# Autodesk Inventor assembly: Main_Solar_Structure
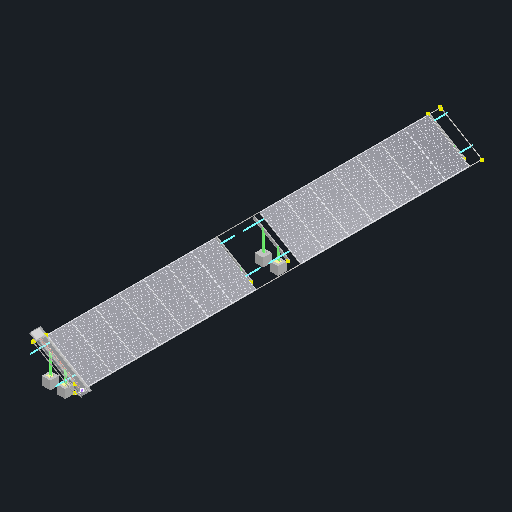
[picture p0: Inventor's stored thumbnail of the model, 512x512]
Saved by Autodesk Inventor 2025.3 (Build 293356030, 356C)
## iProperties
Created: 2019-12-15
Part Number: Main_Solar_Structure
Document SubType Name: Assembly
Designer: Rubens
Sending System: SolidWorks 2021
Last Author: Mohsen
Last Saved: 2022-08-25
Author: Rubens
## Documents named in this file (18)
- C:\Users\Rubens\Downloads\Estrutura Placa - REV00\Solar Mounting Structure\Main_Solar_Structure\Main_Solar_Structure\Estrutura Principal.iam
- C:\Users\Rubens\Downloads\Estrutura Placa - REV00\Solar Mounting Structure\Main_Solar_Structure\Main_Solar_Structure\Small_Column.ipt
- C:\Users\Rubens\Downloads\Estrutura Placa - REV00\Solar Mounting Structure\Main_Solar_Structure\Main_Solar_Structure\Large_Column.ipt
- C:\Users\Rubens\Downloads\Estrutura Placa - REV00\Solar Mounting Structure\Main_Solar_Structure\Main_Solar_Structure\Bottom_Beam.ipt
- C:\Users\Rubens\Downloads\Estrutura Placa - REV00\Solar Mounting Structure\Main_Solar_Structure\Main_Solar_Structure\Top_Beam.iam
- C:\Users\Rubens\Downloads\Estrutura Placa - REV00\Solar Mounting Structure\Main_Solar_Structure\Main_Solar_Structure\Base_Plate.ipt
- C:\Users\Rubens\Downloads\Estrutura Placa - REV00\Solar Mounting Structure\Main_Solar_Structure\Main_Solar_Structure\Base_Support.ipt
- C:\Users\Rubens\Downloads\Estrutura Placa - REV00\Solar Mounting Structure\Main_Solar_Structure\Main_Solar_Structure\Beam_Support.ipt
- C:\Users\Rubens\Downloads\Estrutura Placa - REV00\Solar Mounting Structure\Main_Solar_Structure\Main_Solar_Structure\M10_Screw&Nut.iam
- C:\Users\Rubens\Downloads\Estrutura Placa - REV00\Solar Mounting Structure\Main_Solar_Structure\Main_Solar_Structure\Beam_Connector_Assembly.iam
- C:\Users\Rubens\Downloads\Estrutura Placa - REV00\Solar Mounting Structure\Main_Solar_Structure\Main_Solar_Structure\Base.ipt
- C:\Users\Rubens\Downloads\Estrutura Placa - REV00\Solar Mounting Structure\Main_Solar_Structure\Main_Solar_Structure\ISO - 4034 - M16 - S_.ipt
- C:\Users\Rubens\Downloads\Limpador\MontagemREV0.iam
- C:\Users\Rubens\Downloads\Estrutura Placa - REV00\Solar Mounting Structure\Main_Solar_Structure\Main_Solar_Structure\SolarPV.ipt
- C:\Users\Rubens\Downloads\Estrutura Placa - REV00\Solar Mounting Structure\Main_Solar_Structure\Main_Solar_Structure\Perfil tubo - 30x30x3.ipt
- C:\Users\Rubens\Downloads\Estrutura Placa - REV00\Solar Mounting Structure\Main_Solar_Structure\Main_Solar_Structure\tubo 30 x 30 x 3  - 500.ipt
- C:\Users\Rubens\Downloads\Estrutura Placa - REV00\Solar Mounting Structure\Main_Solar_Structure\Main_Solar_Structure\Limitador.ipt
- C:\Users\Rubens\Downloads\Estrutura Placa - REV00\Solar Mounting Structure\Main_Solar_Structure\Main_Solar_Structure\ISO 12633-2 - 30x30x3 - 2070.ipt
## Components (175 placed, 17 different names)
1. Small_Column:2
2. Base_Plate:2 — Coincidente:15, Coincidente:16, Coincidente:17
3. Base_Plate:4
4. Base_Plate:6
5. Base_Support:3
6. Base_Support:7
7. Base_Support:8
8. Base_Support:9
9. Base_Support:13
10. Base_Support:14
11. Base_Support:15
12. Base_Support:19
13. Base_Support:20
14. Beam_Support:3 — Coincidente:32, Coincidente:33
15. Beam_Support:4 — Coincidente:34, Coincidente:35
16. Beam_Support:5
17. Beam_Support:6
18. Beam_Support:9
19. M10_Screw&Nut:2 [sub-assembly]
20. M10_Screw&Nut:7 [sub-assembly]
21. M10_Screw&Nut:8 [sub-assembly]
22. M10_Screw&Nut:9 [sub-assembly]
23. M10_Screw&Nut:10 [sub-assembly]
24. M10_Screw&Nut:11 [sub-assembly]
25. M10_Screw&Nut:12 [sub-assembly]
26. M10_Screw&Nut:17 [sub-assembly]
27. M10_Screw&Nut:18 [sub-assembly]
28. M10_Screw&Nut:19 [sub-assembly]
29. M10_Screw&Nut:20 [sub-assembly]
30. M10_Screw&Nut:25 [sub-assembly]
31. M10_Screw&Nut:26 [sub-assembly]
32. M10_Screw&Nut:27 [sub-assembly]
33. M10_Screw&Nut:28 [sub-assembly]
34. M10_Screw&Nut:33 [sub-assembly]
35. M10_Screw&Nut:59 [sub-assembly] — Coincidente:63
36. M10_Screw&Nut:60 [sub-assembly]
37. M10_Screw&Nut:61 [sub-assembly]
38. M10_Screw&Nut:62 [sub-assembly]
39. M10_Screw&Nut:63 [sub-assembly]
40. M10_Screw&Nut:64 [sub-assembly]
41. M10_Screw&Nut:65 [sub-assembly]
42. M10_Screw&Nut:66 [sub-assembly]
43. M10_Screw&Nut:67 [sub-assembly]
44. M10_Screw&Nut:68 [sub-assembly]
45. M10_Screw&Nut:69 [sub-assembly]
46. M10_Screw&Nut:71 [sub-assembly] — Coincidente:60
47. M10_Screw&Nut:72 [sub-assembly] — Coincidente:61
48. M10_Screw&Nut:73 [sub-assembly]
49. M10_Screw&Nut:74 [sub-assembly]
50. M10_Screw&Nut:75 [sub-assembly]
51. M10_Screw&Nut:76 [sub-assembly]
52. M10_Screw&Nut:77 [sub-assembly]
53. M10_Screw&Nut:78 [sub-assembly]
54. M10_Screw&Nut:79 [sub-assembly]
55. M10_Screw&Nut:80 [sub-assembly]
56. M10_Screw&Nut:81 [sub-assembly]
57. Beam_Support:24
58. Beam_Support:25
59. Beam_Support:27
60. Beam_Support:28
61. M10_Screw&Nut:90 [sub-assembly]
62. M10_Screw&Nut:91 [sub-assembly]
63. Beam_Connector_Assembly:4 [sub-assembly]
64. ISO - 4034 - M16 - S_:2 — Coincidente:17
65. ISO - 4034 - M16 - S_:43
66. ISO - 4034 - M16 - S_:47
67. ISO - 4034 - M16 - S_:51
68. ISO - 4034 - M16 - S_:55
69. ISO - 4034 - M16 - S_:48
70. ISO - 4034 - M16 - S_:44
71. ISO - 4034 - M16 - S_:56
72. ISO - 4034 - M16 - S_:52
73. ISO - 4034 - M16 - S_:50
74. ISO - 4034 - M16 - S_:46
75. ISO - 4034 - M16 - S_:58
76. ISO - 4034 - M16 - S_:54
77. ISO - 4034 - M16 - S_:49
78. ISO - 4034 - M16 - S_:45
79. ISO - 4034 - M16 - S_:57
80. ISO - 4034 - M16 - S_:53
81. Perfil tubo - 30x30x3:1 — Coincidente:42, Coincidente:43
82. ISO 12633-2 - 30x30x3 - 2070:1 — Coincidente:66, Coincidente:67
83. ISO 12633-2 - 30x30x3 - 2070:2 — Coincidente:68, Alinhado:11, Alinhado:12
84. Base:1 — Coincidente:13, Coincidente:14, Coincidente:16
85. Top_Beam:3 [sub-assembly] — Coincidente:1, Coincidente:2, Coincidente:3, Coincidente:4, Coincidente:33, Alinhado:6, Coincidente:45
86. MontagemREV0:1 [sub-assembly] — Alinhado:1, Coincidente:6, Coincidente:25
87. Perfil tubo - 30x30x3:2 — Coincidente:54, Coincidente:55, Coincidente:56
88. Limitador:1 — Coincidente:53, Coincidente:54
89. SolarPV:1 — Coincidente:1, Alinhado:1, Coincidente:6, Coincidente:19, Coincidente:20, Coincidente:25, Coincidente:42, Coincidente:43
90. Base:2 — Coincidente:13, Coincidente:14
91. Base_Plate:1 — Coincidente:15
92. Base_Support:2
93. Base_Support:1
94. Top_Beam:4 [sub-assembly] — Coincidente:5, Coincidente:31, Coincidente:35, Alinhado:6, Coincidente:58
95. Small_Column:1 — Coincidente:18
96. Bottom_Beam:1 — Coincidente:31, Coincidente:32, Coincidente:34
97. tubo 30 x 30 x 3  - 500:1
98. Limitador:2 — Coincidente:55, Coincidente:56
99. tubo 30 x 30 x 3  - 500:2 — Coincidente:53
100. SolarPV:2 — Coincidente:2, Coincidente:19, Coincidente:20, Coincidente:21, Coincidente:22
101. SolarPV:3 — Coincidente:3, Coincidente:21, Coincidente:22, Coincidente:23, Coincidente:24
102. SolarPV:4 — Coincidente:4, Coincidente:7, Coincidente:8, Coincidente:23, Coincidente:24
103. SolarPV:5 — Coincidente:5, Coincidente:7, Coincidente:8, Coincidente:9, Coincidente:10
104. SolarPV:6 — Coincidente:9, Coincidente:10, Coincidente:11, Coincidente:12
105. SolarPV:7 — Coincidente:11, Coincidente:12, Coincidente:51, Coincidente:52, Coincidente:66, Coincidente:67, Coincidente:68
106. tubo 30 x 30 x 3  - 500:4 — Coincidente:57
107. Perfil tubo - 30x30x3:3 — Coincidente:64, Coincidente:65
108. Bottom_Beam:4 — Coincidente:44, Coincidente:59
109. Perfil tubo - 30x30x3:4 — Coincidente:51
110. tubo 30 x 30 x 3  - 500:3 — Coincidente:52
111. Base:8
112. Base_Support:21
113. Small_Column:4
114. Base_Plate:8
115. Base:6
116. Base:4
117. Beam_Connector_Assembly:6 [sub-assembly]
118. Small_Column:3
119. Bottom_Beam:3
120. Beam_Connector_Assembly:7 [sub-assembly]
121. Beam_Support:10
122. Bottom_Beam:2
123. Beam_Connector_Assembly:5 [sub-assembly]
124. Limitador:3 — Coincidente:57
125. M10_Screw&Nut:58 [sub-assembly] — Coincidente:62
126. Beam_Support:23 — Coincidente:44, Coincidente:45, Coincidente:62, Coincidente:63
127. Beam_Support:26 — Coincidente:58, Coincidente:59, Coincidente:60, Coincidente:61
128. Limitador:4 — Coincidente:64, Coincidente:65
129. Large_Column:1 — Coincidente:18
130. Base:9
131. Top_Beam:5 [sub-assembly]
132. MontagemREV0:2 [sub-assembly]
133. Perfil tubo - 30x30x3:5
134. Limitador:5
135. SolarPV:8 — Alinhado:11, Alinhado:12
136. Base:10
137. Base_Plate:9
138. Base_Support:22
139. Base_Support:23
140. Top_Beam:6 [sub-assembly]
141. Small_Column:5
142. Bottom_Beam:5
143. tubo 30 x 30 x 3  - 500:5
144. Limitador:6
145. tubo 30 x 30 x 3  - 500:6
146. SolarPV:9
147. SolarPV:10
148. SolarPV:11
149. SolarPV:12
150. SolarPV:13
151. SolarPV:14
152. tubo 30 x 30 x 3  - 500:7
153. Perfil tubo - 30x30x3:6
154. Bottom_Beam:6
155. Perfil tubo - 30x30x3:7
156. tubo 30 x 30 x 3  - 500:8
157. Base:11
158. Base_Support:24
159. Small_Column:6
160. Base_Plate:10
161. Base:12
162. Base:13
163. Beam_Connector_Assembly:8 [sub-assembly]
164. Small_Column:7
165. Bottom_Beam:7
166. Beam_Connector_Assembly:9 [sub-assembly]
167. Beam_Support:29
168. Bottom_Beam:8
169. Beam_Connector_Assembly:10 [sub-assembly]
170. Limitador:7
171. M10_Screw&Nut:92 [sub-assembly]
172. Beam_Support:30
173. Beam_Support:31
174. Limitador:8
175. Large_Column:2
## Component patterns: (4 elements, first: Base:1 + Top_Beam:3 + MontagemREV0:1 + Perfil tubo - 30x30x3:2 + Limitador:1 + SolarPV:1 + Base:2 + Base_Plate:1 + Base_Support:2 + Base_Support:1 + Top_Beam:4 + Small_Column:1 + Bottom_Beam:1 + tubo 30 x 30 x 3  - 500:1 + Limitador:2 + tubo 30 x 30 x 3  - 500:2 + SolarPV:2 + SolarPV:3 + SolarPV:4 + SolarPV:5 + SolarPV:6 + SolarPV:7 + tubo 30 x 30 x 3  - 500:4 + Perfil tubo - 30x30x3:3 + Bottom_Beam:4 + Perfil tubo - 30x30x3:4 + tubo 30 x 30 x 3  - 500:3 + Base:8 + Base_Support:21 + Small_Column:4 + Base_Plate:8 + Base:6 + Base:4 + Beam_Connector_Assembly:6 + Small_Column:3 + Bottom_Beam:3 + Beam_Connector_Assembly:7 + Beam_Support:10 + Bottom_Beam:2 + Beam_Connector_Assembly:5 + Limitador:3 + M10_Screw&Nut:58 + Beam_Support:23 + Beam_Support:26 + Limitador:4 + Large_Column:1)
## Relationships (74: Mate 62, Flush 12)
- Coincidente:1 [Mate]: Top_Beam:3 ↔ SolarPV:1
- Coincidente:2 [Mate]: Top_Beam:3 ↔ SolarPV:2
- Coincidente:3 [Mate]: Top_Beam:3 ↔ SolarPV:3
- Coincidente:4 [Mate]: Top_Beam:3 ↔ SolarPV:4
- Coincidente:5 [Mate]: Top_Beam:4 ↔ SolarPV:5
- Alinhado:1 [Flush] (-550 mm): MontagemREV0:1 ↔ SolarPV:1
- Coincidente:6 [Mate] (50 mm): MontagemREV0:1 ↔ SolarPV:1
- Coincidente:7 [Mate]: SolarPV:4 ↔ SolarPV:5
- Coincidente:8 [Mate]: SolarPV:4 ↔ SolarPV:5
- Coincidente:9 [Mate]: SolarPV:5 ↔ SolarPV:6
- Coincidente:10 [Mate]: SolarPV:5 ↔ SolarPV:6
- Coincidente:11 [Mate]: SolarPV:6 ↔ SolarPV:7
- Coincidente:12 [Mate]: SolarPV:6 ↔ SolarPV:7
- Coincidente:13 [Mate] (300 mm): Base:1 ↔ Base:2
- Coincidente:14 [Mate]: Base:1 ↔ Base:2
- Coincidente:15 [Mate]: Base_Plate:2 ↔ Base_Plate:1
- Coincidente:16 [Mate]: Base_Plate:2 ↔ Base:1
- Coincidente:17 [Mate]: Base_Plate:2 ↔ ISO - 4034 - M16 - S_:2
- Coincidente:18 [Mate] (600 mm): Small_Column:1 ↔ Large_Column:1
- Coincidente:19 [Mate]: SolarPV:1 ↔ SolarPV:2
- Coincidente:20 [Mate]: SolarPV:1 ↔ SolarPV:2
- Coincidente:21 [Mate]: SolarPV:2 ↔ SolarPV:3
- Coincidente:22 [Mate]: SolarPV:2 ↔ SolarPV:3
- Coincidente:23 [Mate]: SolarPV:3 ↔ SolarPV:4
- Coincidente:24 [Mate]: SolarPV:3 ↔ SolarPV:4
- Coincidente:25 [Mate]: MontagemREV0:1 ↔ SolarPV:1
- [Mate]: Perfil tubo - 30x30x3:1 ↔ tubo 30 x 30 x 3  - 500:2
- [Mate]: Perfil tubo - 30x30x3:1 ↔ tubo 30 x 30 x 3  - 500:1
- [Flush]: Perfil tubo - 30x30x3:1 ↔ tubo 30 x 30 x 3  - 500:1
- [Flush]: Perfil tubo - 30x30x3:1 ↔ tubo 30 x 30 x 3  - 500:1
- [Mate]: Perfil tubo - 30x30x3:2 ↔ tubo 30 x 30 x 3  - 500:1
- [Flush]: Perfil tubo - 30x30x3:2 ↔ tubo 30 x 30 x 3  - 500:1
- [Mate]: Perfil tubo - 30x30x3:2 ↔ tubo 30 x 30 x 3  - 500:1
- [Mate]: Perfil tubo - 30x30x3:1 ↔ tubo 30 x 30 x 3  - 500:2
- [Flush]: Perfil tubo - 30x30x3:1 ↔ tubo 30 x 30 x 3  - 500:2
- Coincidente:31 [Mate]: Top_Beam:4 ↔ Bottom_Beam:1
- Coincidente:32 [Mate]: Beam_Support:3 ↔ Bottom_Beam:1
- Coincidente:33 [Mate]: Beam_Support:3 ↔ Top_Beam:3
- Coincidente:34 [Mate]: Beam_Support:4 ↔ Bottom_Beam:1
- Coincidente:35 [Mate]: Beam_Support:4 ↔ Top_Beam:4
- Alinhado:6 [Flush]: Top_Beam:3 ↔ Top_Beam:4
- Coincidente:42 [Mate]: Perfil tubo - 30x30x3:1 ↔ SolarPV:1
- Coincidente:43 [Mate]: Perfil tubo - 30x30x3:1 ↔ SolarPV:1
- Coincidente:44 [Mate]: Bottom_Beam:4 ↔ Beam_Support:23
- Coincidente:45 [Mate]: Top_Beam:3 ↔ Beam_Support:23
- [Mate]: tubo 30 x 30 x 3  - 500:4 ↔ Perfil tubo - 30x30x3:3
- [Mate]: Perfil tubo - 30x30x3:3 ↔ tubo 30 x 30 x 3  - 500:3
- [Flush]: Perfil tubo - 30x30x3:3 ↔ tubo 30 x 30 x 3  - 500:3
- [Flush]: Perfil tubo - 30x30x3:3 ↔ tubo 30 x 30 x 3  - 500:3
- [Mate]: Perfil tubo - 30x30x3:4 ↔ tubo 30 x 30 x 3  - 500:3
- [Flush]: Perfil tubo - 30x30x3:4 ↔ tubo 30 x 30 x 3  - 500:3
- [Mate]: Perfil tubo - 30x30x3:4 ↔ tubo 30 x 30 x 3  - 500:3
- [Mate]: tubo 30 x 30 x 3  - 500:4 ↔ Perfil tubo - 30x30x3:3
- [Flush]: tubo 30 x 30 x 3  - 500:4 ↔ Perfil tubo - 30x30x3:3
- Coincidente:51 [Mate]: SolarPV:7 ↔ Perfil tubo - 30x30x3:4
- Coincidente:52 [Mate]: SolarPV:7 ↔ tubo 30 x 30 x 3  - 500:3
- Coincidente:53 [Mate]: Limitador:1 ↔ tubo 30 x 30 x 3  - 500:2
- Coincidente:54 [Mate]: Perfil tubo - 30x30x3:2 ↔ Limitador:1
- Coincidente:55 [Mate]: Perfil tubo - 30x30x3:2 ↔ Limitador:2
- Coincidente:56 [Mate]: Perfil tubo - 30x30x3:2 ↔ Limitador:2
- Coincidente:57 [Mate]: tubo 30 x 30 x 3  - 500:4 ↔ Limitador:3
- Coincidente:58 [Mate]: Top_Beam:4 ↔ Beam_Support:26
- Coincidente:59 [Mate]: Bottom_Beam:4 ↔ Beam_Support:26
- Coincidente:60 [Mate]: M10_Screw&Nut:71 ↔ Beam_Support:26
- Coincidente:61 [Mate]: M10_Screw&Nut:72 ↔ Beam_Support:26
- Coincidente:62 [Mate]: M10_Screw&Nut:58 ↔ Beam_Support:23
- Coincidente:63 [Mate]: M10_Screw&Nut:59 ↔ Beam_Support:23
- Coincidente:64 [Mate]: Perfil tubo - 30x30x3:3 ↔ Limitador:4
- Coincidente:65 [Mate]: Perfil tubo - 30x30x3:3 ↔ Limitador:4
- Coincidente:66 [Mate]: ISO 12633-2 - 30x30x3 - 2070:1 ↔ SolarPV:7
- Coincidente:67 [Mate]: ISO 12633-2 - 30x30x3 - 2070:1 ↔ SolarPV:7
- Coincidente:68 [Mate]: ISO 12633-2 - 30x30x3 - 2070:2 ↔ SolarPV:7
- Alinhado:11 [Flush]: ISO 12633-2 - 30x30x3 - 2070:2 ↔ SolarPV:8
- Alinhado:12 [Flush]: ISO 12633-2 - 30x30x3 - 2070:2 ↔ SolarPV:8
## Named parameters: d92_d72 = 0 mm, d93_d73 = 0 mm, d94_d74 = 0 mm, d95_d75 = 0 mm, d96_d76 = 0 mm, d97_d77 = 0 mm, d98_d79 = 0 mm, d99_d80 = 0 mm, d100_d81 = 0 mm
